# Autodesk Inventor assembly: Rosses spaces and ball screw bearing
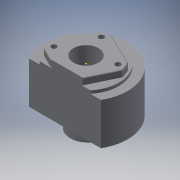
[picture p0: Inventor's stored thumbnail of the model, 180x180]
Saved by Autodesk Inventor 2018 (Build 220112000, 112)
## iProperties
Created: 2017-07-25
Part Number: Rosses spaces and ball screw bearing
Document SubType Name: Assembly
Designer: M227562
Author: M227562
## Documents named in this file (3)
- C:\Users\P301319\Documents\GitHub\CNC-Lathe-CAD\Archive\X Axis Nut Correct\Rosses spaces and ball screw bearing.iam
- C:\Users\P301319\Documents\GitHub\CNC-Lathe-CAD\Archive\X Axis Nut Correct\608ZZ Ball Screw Support Unit.ipt
- C:\Users\P301319\Documents\GitHub\CNC-Lathe-CAD\Archive\X Axis Nut Correct\Ross Made spacer.ipt
## Components (2 placed, 2 different names)
1. 608ZZ Ball Screw Support Unit:1 — Mate:1, Mate:2
2. Ross Made spacer:1 — Mate:1, Mate:2
## Relationships (2: Mate 2)
- Mate:1: 608ZZ Ball Screw Support Unit:1 ↔ Ross Made spacer:1
- Mate:2: 608ZZ Ball Screw Support Unit:1 ↔ Ross Made spacer:1
